# Autodesk Inventor assembly: buttons
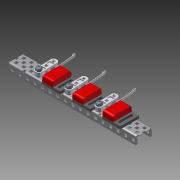
[picture p0: Inventor's stored thumbnail of the model, 180x180]
Saved by Autodesk Inventor 2014 SP1 (Build 180222100, 222)
## iProperties
Created: 2014-03-19
Part Number: buttons
Document SubType Name: Assembly
Designer: Ryan
Author: Ryan
## Documents named in this file (7)
- C:\Users\Ryan\Desktop\sw\toss up 4th robot\buttons.iam
- C:\Users\Ryan\Desktop\sw\lib\Super Sonic Sparks VEX CAD Library\Motors & Sensors\Limit Switch (Sensor).iam
- C:\Users\Ryan\Desktop\sw\lib\Aperture VEX CAD Library\Bearing Blocks\Bearing Block.ipt
- C:\Users\Ryan\Desktop\sw\lib\Aperture VEX CAD Library\Spacers\thin\SPACER-0320-00625.ipt
- C:\Users\Ryan\Desktop\sw\lib\Aperture VEX CAD Library\Hardware\8-32\8-32_.500.ipt
- C:\Users\Ryan\Desktop\sw\lib\Aperture VEX CAD Library\Hardware\8-32\8-32 nylock.ipt
- C:\Users\Ryan\Desktop\sw\lib\Aperture VEX CAD Library\Metal\C Channel\2 x 17_actual.ipt
## Components (16 placed, 6 different names)
1. 2 x 17_actual:1 — Mate:13, Mate:14, Mate:15, Mate:16, Mate:17, Mate:18, Mate:19
2. Limit Switch (Sensor):1 [sub-assembly] — Mate:13, Mate:14, Mate:15
3. 8-32_.500:1 — Mate:10, Mate:11, Mate:16, Mate:19
4. 8-32 nylock:1 — Mate:11, Mate:12
5. Bearing Block:1 — Mate:4, Mate:5, Mate:12
6. SPACER-0320-00625:1 — Mate:4, Mate:5, Mate:10, Mate:17, Mate:18
7. Limit Switch (Sensor):2 [sub-assembly]
8. 8-32_.500:2
9. 8-32 nylock:2
10. Bearing Block:2
11. SPACER-0320-00625:2
12. Limit Switch (Sensor):3 [sub-assembly]
13. 8-32_.500:3
14. 8-32 nylock:3
15. Bearing Block:3
16. SPACER-0320-00625:3
## Component patterns: (3 elements, first: Limit Switch (Sensor):1 + 8-32_.500:1 + 8-32 nylock:1 + Bearing Block:1 + SPACER-0320-00625:1)
## Relationships (12: Mate 12)
- Mate:4: Bearing Block:1 ↔ SPACER-0320-00625:1
- Mate:5: Bearing Block:1 ↔ SPACER-0320-00625:1
- Mate:10: 8-32_.500:1 ↔ SPACER-0320-00625:1
- Mate:11: 8-32_.500:1 ↔ 8-32 nylock:1
- Mate:12: 8-32 nylock:1 ↔ Bearing Block:1
- Mate:13: 2 x 17_actual:1 ↔ Limit Switch (Sensor):1
- Mate:14 (2.3114 mm): 2 x 17_actual:1 ↔ Limit Switch (Sensor):1
- Mate:15 (-12.7 mm): 2 x 17_actual:1 ↔ Limit Switch (Sensor):1
- Mate:16 (2.3114 mm): 2 x 17_actual:1 ↔ 8-32_.500:1
- Mate:17: 2 x 17_actual:1 ↔ SPACER-0320-00625:1
- Mate:18 (2.3114 mm): 2 x 17_actual:1 ↔ SPACER-0320-00625:1
- Mate:19: 2 x 17_actual:1 ↔ 8-32_.500:1
## Named parameters: q = 2.3114 mm
